# Autodesk Inventor assembly: Application_Discovery_Kit_Extension_Interferometer_Michelson
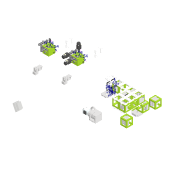
[picture p0: Inventor's stored thumbnail of the model, 180x180]
Saved by Autodesk Inventor 2022 (Build 260153000, 153)
## iProperties
Created: 2022-10-31
Part Number: Application_Discovery_Kit_Extension_Interferometer_Michelson
Document SubType Name: Assembly
Designer: UC2
Author: UC2
## Documents named in this file (18)
- C:\Users\UC2\Documents\GitHub\openUC2-Hackathon-openOCTRemote\INVENTOR\Application_Hackathon_openOCT.iam
- C:\Users\UC2\Documents\GitHub\openUC2-Hackathon-openOCTRemote\INVENTOR\Assembly_Cube_Kinematic_Mirrormount_Astromedia_30x40x1_45_PRO_magnetic.iam
- C:\Users\UC2\Documents\GitHub\openUC2-Hackathon-openOCTRemote\INVENTOR\Assembly_Cube_Kinematic_Mirrormount_Astromedia_30x40x1_90_PRO_magnetic.iam
- C:\Users\UC2\Documents\GitHub\openUC2-Hackathon-openOCTRemote\INVENTOR\Assembly_Cube_empty_IM_v3.iam
- C:\Users\UC2\Documents\GitHub\openUC2-Hackathon-openOCTRemote\INVENTOR\Assembly_Cube_Beamsplitter_Astromedia_Partiallytransparent_30x40x1mmv3.iam
- C:\Users\UC2\Documents\GitHub\openUC2-Hackathon-openOCTRemote\INVENTOR\Assembly_Cube_Lens_holder_25mm_v3.iam
- C:\Users\UC2\Documents\GitHub\openUC2-Hackathon-openOCTRemote\INVENTOR\10_Base_puzzle_v3.ipt
- C:\Users\UC2\Documents\GitHub\openUC2-Hackathon-openOCTRemote\INVENTOR\Assembly_Cube_Kinematic_Mirrormount_Thorlabs_45_PRO_v3.iam
- C:\Users\UC2\Documents\GitHub\openUC2-Hackathon-openOCTRemote\INVENTOR\Assembly_Cube_Kinematic_Mirrormount_Thorlabs_90_PRO_magnetic_v3.iam
- C:\Users\UC2\Documents\GitHub\openUC2-Hackathon-openOCTRemote\INVENTOR\Assembly_XYZ_Stage_Micrometer_lightsheet.iam
- C:\Users\UC2\Documents\GitHub\openUC2-Hackathon-openOCTRemote\INVENTOR\Assembly_XYZ_Stage_Micrometer_lightsheet_manual.iam
- C:\Users\UC2\Documents\GitHub\openUC2-Hackathon-openOCTRemote\INVENTOR\20_Cube_Insert_Laser_Holder_fixed_v3.ipt
- C:\Users\UC2\Documents\GitHub\openUC2-Hackathon-openOCTRemote\INVENTOR\20_Cube_Insert_Lasertack_mount_v3.ipt
- C:\Users\UC2\Documents\GitHub\openUC2-Hackathon-openOCTRemote\INVENTOR\Assembly_Cube_Lens_holder_Thorlabs_AC254_v3.iam
- C:\Users\UC2\Documents\GitHub\openUC2-Hackathon-openOCTRemote\INVENTOR\Assembly_Cube_Berrybase_CCTVLens_100mm.iam
- C:\Users\UC2\Desktop\OCT_Jenny\Cube_Insert_Motion_adapter_srew_back.ipt
- C:\Users\UC2\Desktop\OCT_Jenny\Cube_Insert_Motion_adapter_srew.ipt
- C:\Users\UC2\Desktop\OCT_Jenny\OCT_SpiegelAdapter_MovingSt..ipt
## Components (38 placed, 17 different names)
1. Assembly_Cube_Kinematic_Mirrormount_Astromedia_30x40x1_45_PRO_magnetic:1 [sub-assembly] — Passend:7, Passend:8, Fluchtend:7, Fluchtend:11, Fluchtend:12
2. Assembly_Cube_Kinematic_Mirrormount_Astromedia_30x40x1_90_PRO_magnetic:1 [sub-assembly] — Fluchtend:15, Passend:11, Fluchtend:16, Fluchtend:18
3. Assembly_Cube_Kinematic_Mirrormount_Astromedia_30x40x1_90_PRO_magnetic:2 [sub-assembly] — Passend:10, Fluchtend:13, Fluchtend:14, Fluchtend:16, Fluchtend:17
4. Assembly_Cube_empty_IM_v3:1 [sub-assembly] — Fluchtend:5, Passend:6
5. Assembly_Cube_Beamsplitter_Astromedia_Partiallytransparent_30x40x1mmv3:1 [sub-assembly] — Passend:9, Fluchtend:11, Fluchtend:12, Fluchtend:13, Fluchtend:14, Fluchtend:15
6. Assembly_Cube_empty_IM_v3:2 [sub-assembly] — Fluchtend:17, Passend:12, Fluchtend:18
7. Assembly_Cube_Kinematic_Mirrormount_Thorlabs_45_PRO_v3:1 [sub-assembly]
8. Assembly_Cube_Kinematic_Mirrormount_Thorlabs_90_PRO_magnetic_v3:1 [sub-assembly]
9. Assembly_XYZ_Stage_Micrometer_lightsheet:1 [sub-assembly]
10. Assembly_XYZ_Stage_Micrometer_lightsheet_manual:1 [sub-assembly]
11. 20_Cube_Insert_Laser_Holder_fixed_v3:1
12. 20_Cube_Insert_Lasertack_mount_v3:1
13. Assembly_Cube_Lens_holder_Thorlabs_AC254_v3:1 [sub-assembly]
14. Assembly_Cube_Lens_holder_Thorlabs_AC254_v3:2 [sub-assembly]
15. Assembly_Cube_Berrybase_CCTVLens_100mm:1 [sub-assembly]
16. Cube_Insert_Motion_adapter_srew_back:1
17. Cube_Insert_Motion_adapter_srew:1
18. OCT_SpiegelAdapter_MovingSt.:1
19. Assembly_Cube_Lens_holder_25mm_v3:2 [sub-assembly] — Fluchtend:3, Passend:5
20. Assembly_Cube_Lens_holder_25mm_v3:3 [sub-assembly] — Fluchtend:5, Passend:7
21. 10_Base_puzzle_v3:6 — Fluchtend:8, Fluchtend:9, Fluchtend:10, Passend:9
22. 10_Base_puzzle_v3:7 — Passend:11
23. 10_Base_puzzle_v3:8 — Passend:10
24. 10_Base_puzzle_v3:9 — Passend:12
25. 10_Base_puzzle_v3:1 — Passend:1, Passend:2, Passend:3, Passend:8, Fluchtend:7, Fluchtend:9, Fluchtend:10
26. 10_Base_puzzle_v3:2 — Fluchtend:8
27. 10_Base_puzzle_v3:3 — Passend:5, Passend:6
28. 10_Base_puzzle_v3:4 — Fluchtend:3
29. 10_Base_puzzle_v3:5
30. 10_Base_puzzle_v3:10
31. 10_Base_puzzle_v3:11
32. 10_Base_puzzle_v3:12
33. 10_Base_puzzle_v3:13
34. 10_Base_puzzle_v3:14
35. 10_Base_puzzle_v3:15
36. 10_Base_puzzle_v3:16
37. 10_Base_puzzle_v3:17
38. 10_Base_puzzle_v3:18
## Component patterns: (2 elements, first: Assembly_Cube_Lens_holder_25mm_v3:2), (2 elements), (4 elements, first: 10_Base_puzzle_v3:6), (5 elements, first: 10_Base_puzzle_v3:1), Komponentenanordnung 3:2 (4 elements), Komponentenanordnung 1:2 (5 elements)
## Relationships (25: Flush 14, Mate 11)
- Passend:1 [Mate]: 10_Base_puzzle_v3:1
- Passend:2 [Mate]: 10_Base_puzzle_v3:1
- Passend:3 [Mate]: 10_Base_puzzle_v3:1
- Fluchtend:3 [Flush]: Assembly_Cube_Lens_holder_25mm_v3:2 ↔ 10_Base_puzzle_v3:4
- Passend:5 [Mate]: Assembly_Cube_Lens_holder_25mm_v3:2 ↔ 10_Base_puzzle_v3:3
- Fluchtend:5 [Flush]: Assembly_Cube_empty_IM_v3:1 ↔ Assembly_Cube_Lens_holder_25mm_v3:3
- Passend:6 [Mate]: Assembly_Cube_empty_IM_v3:1 ↔ 10_Base_puzzle_v3:3
- Passend:7 [Mate]: Assembly_Cube_Kinematic_Mirrormount_Astromedia_30x40x1_45_PRO_magnetic:1 ↔ Assembly_Cube_Lens_holder_25mm_v3:3
- Passend:8 [Mate]: Assembly_Cube_Kinematic_Mirrormount_Astromedia_30x40x1_45_PRO_magnetic:1 ↔ 10_Base_puzzle_v3:1
- Fluchtend:7 [Flush]: Assembly_Cube_Kinematic_Mirrormount_Astromedia_30x40x1_45_PRO_magnetic:1 ↔ 10_Base_puzzle_v3:1
- Fluchtend:8 [Flush] (50 mm): 10_Base_puzzle_v3:6 ↔ 10_Base_puzzle_v3:2
- Fluchtend:9 [Flush]: 10_Base_puzzle_v3:6 ↔ 10_Base_puzzle_v3:1
- Fluchtend:10 [Flush]: 10_Base_puzzle_v3:6 ↔ 10_Base_puzzle_v3:1
- Passend:9 [Mate]: Assembly_Cube_Beamsplitter_Astromedia_Partiallytransparent_30x40x1mmv3:1 ↔ 10_Base_puzzle_v3:6
- Fluchtend:11 [Flush] (-50 mm): Assembly_Cube_Kinematic_Mirrormount_Astromedia_30x40x1_45_PRO_magnetic:1 ↔ Assembly_Cube_Beamsplitter_Astromedia_Partiallytransparent_30x40x1mmv3:1
- Fluchtend:12 [Flush]: Assembly_Cube_Kinematic_Mirrormount_Astromedia_30x40x1_45_PRO_magnetic:1 ↔ Assembly_Cube_Beamsplitter_Astromedia_Partiallytransparent_30x40x1mmv3:1
- Passend:10 [Mate]: Assembly_Cube_Kinematic_Mirrormount_Astromedia_30x40x1_90_PRO_magnetic:2 ↔ 10_Base_puzzle_v3:8
- Fluchtend:13 [Flush] (-50 mm): Assembly_Cube_Kinematic_Mirrormount_Astromedia_30x40x1_90_PRO_magnetic:2 ↔ Assembly_Cube_Beamsplitter_Astromedia_Partiallytransparent_30x40x1mmv3:1
- Fluchtend:14 [Flush]: Assembly_Cube_Kinematic_Mirrormount_Astromedia_30x40x1_90_PRO_magnetic:2 ↔ Assembly_Cube_Beamsplitter_Astromedia_Partiallytransparent_30x40x1mmv3:1
- Fluchtend:15 [Flush] (50 mm): Assembly_Cube_Kinematic_Mirrormount_Astromedia_30x40x1_90_PRO_magnetic:1 ↔ Assembly_Cube_Beamsplitter_Astromedia_Partiallytransparent_30x40x1mmv3:1
- Passend:11 [Mate]: Assembly_Cube_Kinematic_Mirrormount_Astromedia_30x40x1_90_PRO_magnetic:1 ↔ 10_Base_puzzle_v3:7
- Fluchtend:16 [Flush] (50 mm): Assembly_Cube_Kinematic_Mirrormount_Astromedia_30x40x1_90_PRO_magnetic:1 ↔ Assembly_Cube_Kinematic_Mirrormount_Astromedia_30x40x1_90_PRO_magnetic:2
- Fluchtend:17 [Flush]: Assembly_Cube_Kinematic_Mirrormount_Astromedia_30x40x1_90_PRO_magnetic:2 ↔ Assembly_Cube_empty_IM_v3:2
- Passend:12 [Mate]: Assembly_Cube_empty_IM_v3:2 ↔ 10_Base_puzzle_v3:9
- Fluchtend:18 [Flush]: Assembly_Cube_Kinematic_Mirrormount_Astromedia_30x40x1_90_PRO_magnetic:1 ↔ Assembly_Cube_empty_IM_v3:2
